# Autodesk Inventor assembly: Assembly1
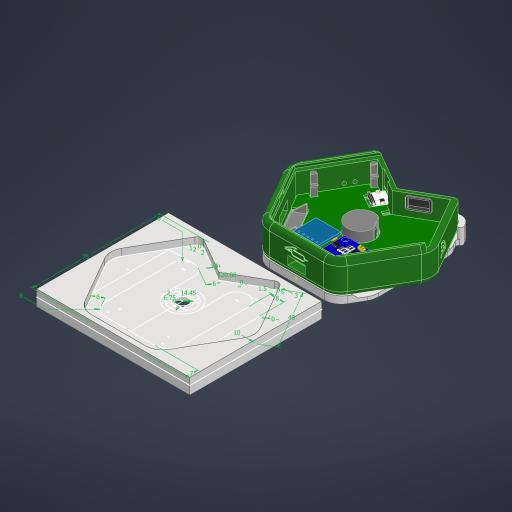
[picture p0: Inventor's stored thumbnail of the model, 512x512]
Saved by Autodesk Inventor 2023 (Build 270158000, 158)
## iProperties
Created: 2022-06-22
Part Number: Assembly1
Document SubType Name: Assembly
Designer: jevan
Author: jevan
## Documents named in this file (14)
- C:\Users\jevan\Documents\Assembly1.iam
- C:\Users\jevan\Documents\LilypadShellProto1.ipt
- C:\Users\jevan\Downloads\wemos-d1-mini-with-pin-header-1.snapshot.1\WEMOS-D1-mini.ipt
- C:\Users\jevan\Documents\LilypadLidProto1.ipt
- C:\Users\jevan\Documents\Models\Lilypad\LilypadTrayProto.ipt
- C:\Users\jevan\Documents\Models\capteur-gyroscopique-analogique-accelerometre-3-axes-mpu-6050-1.snapshot.2\MPU-6050\MPU-6050.ipt
- C:\Users\jevan\Documents\Models\tp4056-charging-module-type-c-1.snapshot.1\TP4056_Charging_Module_Type_C.ipt
- C:\Users\jevan\Documents\Models\Lilypad\503759.ipt
- C:\Users\jevan\Documents\Models\Lilypad\LilypadPCB.ipt
- C:\Users\jevan\Documents\Models\mpu-9250-9dof-imu-1.snapshot.4\MPU-9250.iam
- C:\Users\jevan\Documents\Models\gy-271-hmc5883l-triple-3-axis-digital-compass-magnetometer-sensor-module-1.snapshot.3\GY-271 HMC5883L Triple 3 Axis Digital Compass.ipt
- C:\Users\jevan\Documents\Models\Lilypad\LilypadClipProto.ipt
- C:\Users\jevan\Documents\Models\Lilypad\LilypadCover.ipt
- C:\Users\jevan\Documents\Models\Lilypad\V4\CalibrationBlockV3.ipt
## Components (13 placed, 13 different names)
1. LilypadShellProto1:1 — Mate:2, Mate:3, Mate:17, Flush:6, Flush:7, Flush:8, Mate:23, Mate:24, Mate:25, Mate:26, Flush:9
2. WEMOS-D1-mini:1 — Mate:11, Mate:16, Mate:17
3. LilypadLidProto1:1 — Mate:2, Mate:26
4. LilypadTrayProto:1 — Mate:3, Mate:11, Mate:12, Mate:13, Mate:14, Mate:16, Flush:4, Mate:25
5. MPU-6050:1
6. TP4056_Charging_Module_Type_C:1 — Flush:1, Mate:15, Flush:5
7. 503759:1 — Mate:14
8. LilypadPCB:1 — Mate:12, Mate:13, Flush:1, Mate:15, Mate:18, Mate:20, Flush:3, Flush:4, Mate:21, Flush:5
9. MPU-9250:1 [sub-assembly] — Mate:19, Mate:20, Flush:2, Flush:3
10. GY-271 HMC5883L Triple 3 Axis Digital Compass:1 — Mate:18, Mate:19, Flush:2, Mate:21
11. LilypadClipProto:1 — Flush:6, Flush:8
12. LilypadCover:1 — Flush:7, Mate:23, Mate:24
13. CalibrationBlockV3:1 — Flush:9
## Relationships (26: Mate 17, Flush 9)
- Mate:2 (-0.05 mm): LilypadShellProto1:1 ↔ LilypadLidProto1:1
- Mate:3: LilypadShellProto1:1 ↔ LilypadTrayProto:1
- Mate:11: WEMOS-D1-mini:1 ↔ LilypadTrayProto:1
- Mate:12 (0.45 mm): LilypadTrayProto:1 ↔ LilypadPCB:1
- Mate:13: LilypadTrayProto:1 ↔ LilypadPCB:1
- Mate:14: LilypadTrayProto:1 ↔ 503759:1
- Flush:1: TP4056_Charging_Module_Type_C:1 ↔ LilypadPCB:1
- Mate:15 (1.56 mm): TP4056_Charging_Module_Type_C:1 ↔ LilypadPCB:1
- Mate:16 (1 mm): WEMOS-D1-mini:1 ↔ LilypadTrayProto:1
- Mate:17: LilypadShellProto1:1 ↔ WEMOS-D1-mini:1
- Mate:18 (2.4 mm): LilypadPCB:1 ↔ GY-271 HMC5883L Triple 3 Axis Digital Compass:1
- Mate:19 (0.75 mm): MPU-9250:1 ↔ GY-271 HMC5883L Triple 3 Axis Digital Compass:1
- Mate:20: LilypadPCB:1 ↔ MPU-9250:1
- Flush:2: MPU-9250:1 ↔ GY-271 HMC5883L Triple 3 Axis Digital Compass:1
- Flush:3 (9.2 mm): LilypadPCB:1 ↔ MPU-9250:1
- Flush:4: LilypadTrayProto:1 ↔ LilypadPCB:1
- Mate:21: LilypadPCB:1 ↔ GY-271 HMC5883L Triple 3 Axis Digital Compass:1
- Flush:5: TP4056_Charging_Module_Type_C:1 ↔ LilypadPCB:1
- Flush:6: LilypadShellProto1:1 ↔ LilypadClipProto:1
- Flush:7: LilypadShellProto1:1 ↔ LilypadCover:1
- Flush:8: LilypadShellProto1:1 ↔ LilypadClipProto:1
- Mate:23: LilypadShellProto1:1 ↔ LilypadCover:1
- Mate:24: LilypadShellProto1:1 ↔ LilypadCover:1
- Mate:25: LilypadShellProto1:1 ↔ LilypadTrayProto:1
- Mate:26: LilypadShellProto1:1 ↔ LilypadLidProto1:1
- Flush:9: LilypadShellProto1:1 ↔ CalibrationBlockV3:1
